# Autodesk Inventor assembly: 110-03
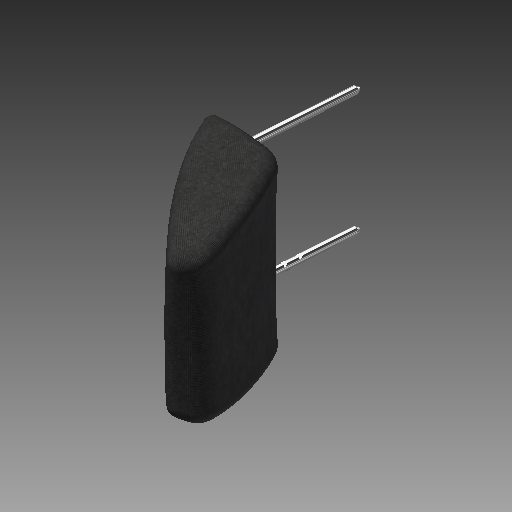
[picture p0: Inventor's stored thumbnail of the model, 512x512]
Saved by Autodesk Inventor 2019 (Build 230136000, 136)
## iProperties
Company: Autodesk Inc.
Created: 2007-12-28
Part Number: 110-03
Document SubType Name: Assembly
Designer: Autodesk Inc.
Mass: 3981.2 g
Surface Area: 4595.07 cm^2
Volume: 3706.53 cm^3
Density: 1.0741 g/cm^3
Description: HEAD REST ASSEMBLY
Component Category: Head Rest
Author: Inventor
## Documents named in this file (4)
- C:\TEMP\Car Seat\Workspace\Headrest.iam
- C:\TEMP\Car Seat\Workspace\Headrest Bar.ipt
- C:\TEMP\Car Seat\Workspace\Headrest Cushion.ipt
- C:\TEMP\Car Seat\Workspace\Headrest Cover.ipt
## Components (3 placed, 3 different names)
1. Headrest Bar:1 — Flush:1, Flush:2, Mate:1
2. Headrest Cushion:1 — Flush:1, Flush:2, Flush:3, Flush:4, Flush:5, Mate:1
3. Headrest Cover:1 — Flush:3, Flush:4, Flush:5
## Relationships (6: Flush 5, Mate 1)
- Flush:1: Headrest Bar:1 ↔ Headrest Cushion:1
- Flush:2 (166 mm): Headrest Bar:1 ↔ Headrest Cushion:1
- Flush:3: Headrest Cushion:1 ↔ Headrest Cover:1
- Flush:4: Headrest Cushion:1 ↔ Headrest Cover:1
- Flush:5: Headrest Cushion:1 ↔ Headrest Cover:1
- Mate:1 (-126.3 mm): Headrest Bar:1 ↔ Headrest Cushion:1
